# Autodesk Inventor assembly: assembly
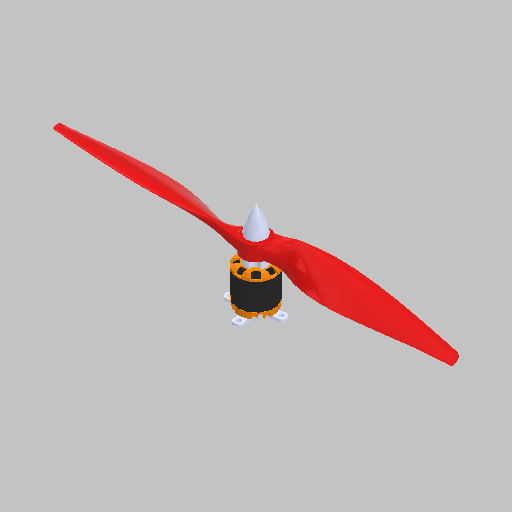
[picture p0: Inventor's stored thumbnail of the model, 512x512]
Saved by Autodesk Inventor 2025.2 (Build 292293000, 293)
## iProperties
Created: 2014-10-30
Part Number: assembly
Document SubType Name: Assembly
Designer: phmca
Sending System: SolidWorks 2013
Last Author: Micheal
Last Saved: 2014-10-30
Author: phmca
## Documents named in this file (8)
- C:\Users\phmca\OneDrive\Documentos\TCC\TCC\brushless-motor-with-prop-1.snapshot.1\assembly\assembly.iam
- C:\Users\phmca\OneDrive\Documentos\TCC\TCC\brushless-motor-with-prop-1.snapshot.1\assembly\cylinderBody.ipt
- C:\Users\phmca\OneDrive\Documentos\TCC\TCC\brushless-motor-with-prop-1.snapshot.1\assembly\motorBase.ipt
- C:\Users\phmca\OneDrive\Documentos\TCC\TCC\brushless-motor-with-prop-1.snapshot.1\assembly\mount.ipt
- C:\Users\phmca\OneDrive\Documentos\TCC\TCC\brushless-motor-with-prop-1.snapshot.1\assembly\motorTop.ipt
- C:\Users\phmca\OneDrive\Documentos\TCC\TCC\brushless-motor-with-prop-1.snapshot.1\assembly\propSpool.ipt
- C:\Users\phmca\OneDrive\Documentos\TCC\TCC\brushless-motor-with-prop-1.snapshot.1\assembly\APC 12x6.ipt
- C:\Users\phmca\OneDrive\Documentos\TCC\TCC\brushless-motor-with-prop-1.snapshot.1\assembly\propTop.ipt
## Components (7 placed, 7 different names)
1. cylinderBody:1
2. motorBase:1
3. mount:1 — Coincidente:1, Ângulo:1, Coincidente:3, Coincidente:4, Coincidente:7, Ângulo:3, Coincidente:10, Ângulo:4
4. motorTop:1
5. propSpool:1
6. APC 12x6:1
7. propTop:1
## Relationships (14: Mate 11, Angle 3)
- Coincidente:1 [Mate]: mount:1
- Ângulo:1 [Angle] (0 deg): mount:1
- Coincidente:3 [Mate]: mount:1
- Coincidente:4 [Mate]: mount:1
- Coincidente:5 [Mate]
- Coincidente:6 [Mate]
- Coincidente:7 [Mate]: mount:1
- Coincidente:8 [Mate]
- Coincidente:9 [Mate]
- Ângulo:3 [Angle] (0 deg): mount:1
- Coincidente:10 [Mate]: mount:1
- Coincidente:11 [Mate]
- Coincidente:12 [Mate]
- Ângulo:4 [Angle] (0 deg): mount:1
